# Autodesk Inventor assembly: Lime Extruder - ASM
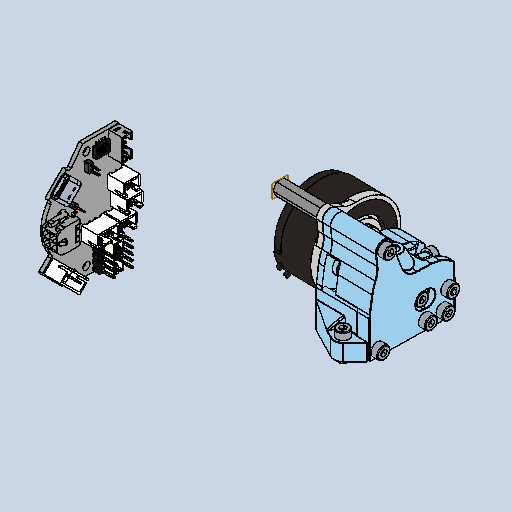
[picture p0: Inventor's stored thumbnail of the model, 512x512]
Saved by Autodesk Inventor 2026 (Build 300175050, 175E)
## iProperties
Created: 2025-07-30
Part Number: Lime Extruder - ASM
Description: STEP AP242
Document SubType Name: Assembly
Designer: tdxt
Sending System: ONSHAPE BY PTC INC, 1.201
Preprocessor: ST-DEVELOPER v20
Title: 688046dff3c7ef29f6bbb4df
## Documents named in this file (12)
- D:\Github\Lime\Lime Extruder - ASM\Lime Extruder - ASM\Lime Extruder - ASM.iam
- D:\Github\Lime\Lime Extruder - ASM\Lime Extruder - ASM\GEAR_7MM_12_TEETH_0_5_3MM_BORE.ipt
- D:\Github\Lime\Lime Extruder - ASM\Lime Extruder - ASM\Hex socket head cap screw M3x0.50 x 20.ipt
- D:\Github\Lime\Lime Extruder - ASM\Lime Extruder - ASM\Hex socket head cap screw M3x0.50 x 10.ipt
- D:\Github\Lime\Lime Extruder - ASM\Lime Extruder - ASM\Idler Arm.ipt
- D:\Github\Lime\Lime Extruder - ASM\Lime Extruder - ASM\Hex socket head cap screw M3x0.50 x 30.ipt
- D:\Github\Lime\Lime Extruder - ASM\Lime Extruder - ASM\Front Frame.ipt
- D:\Github\Lime\Lime Extruder - ASM\Lime Extruder - ASM\K1_EXTRUDER_MOTOR_-_MOONS_CSE14.ipt
- D:\Github\Lime\Lime Extruder - ASM\Lime Extruder - ASM\Back Frame.ipt
- D:\Github\Lime\Lime Extruder - ASM\hex spacer standoff nut_M3 L20\hex spacer standoff nut_M3 L20\hex spacer standoff nut_M3 L20.ipt
- D:\Github\Lime\Lime Extruder - ASM\EBB36 v4\EBB36 v4\EBB36 v4.ipt
- D:\Github\Lime\Lime Extruder - ASM\Lime Extruder - ASM\CAN Board Holder.ipt
## Components (18 placed, 17 different names)
1. Idler Arm — 旋转:6, 旋转:14
2. Front Plate — 旋转:2, 旋转:3, 旋转:7, 旋转:9, 旋转:10, 旋转:11, 旋转:12, 旋转:13
3. Back Plate — 旋转:2, 旋转:3, 旋转:4, 旋转:5, 旋转:6, 刚性:1, 旋转:8
4. EBB36 v4:1
5. CAN Board Holder:1 — 表面齐平:1
6. NAUO1 — 旋转:1
7. NAUO11 — 旋转:1, 旋转:4, 旋转:5, 插入:1, 插入:2
8. hex spacer standoff nut_M3 L20:1 — 插入:2
9. hex spacer standoff nut_M3 L20:2 — 插入:1, 表面齐平:1
10. NAUO2 — 旋转:11
11. NAUO5 — 旋转:9
12. NAUO13 — 旋转:10
13. NAUO3 — 旋转:14
14. NAUO7 — 刚性:1
15. NAUO8 — 旋转:12
16. NAUO9 — 旋转:13
17. NAUO10 — 旋转:7
18. NAUO12 — 旋转:8
## Relationships (18: RevoluteJoint 14, Insert 2, WeldJoint 1, Flush 1)
- 旋转:1 [RevoluteJoint]: NAUO1 ↔ NAUO11
- 旋转:2 [RevoluteJoint] (-0.1 mm): Front Plate ↔ Back Plate
- 旋转:3 [RevoluteJoint] (0.2 mm): Front Plate ↔ Back Plate
- 旋转:4 [RevoluteJoint]: Back Plate ↔ NAUO11
- 旋转:5 [RevoluteJoint]: Back Plate ↔ NAUO11
- 旋转:6 [RevoluteJoint] (0.2 mm): Idler Arm ↔ Back Plate
- 旋转:7 [RevoluteJoint] (3 mm): Front Plate ↔ NAUO10
- 刚性:1 [WeldJoint]: Back Plate ↔ NAUO7
- 旋转:8 [RevoluteJoint]: Back Plate ↔ NAUO12
- 旋转:9 [RevoluteJoint]: Front Plate ↔ NAUO5
- 旋转:10 [RevoluteJoint]: Front Plate ↔ NAUO13
- 旋转:11 [RevoluteJoint]: Front Plate ↔ NAUO2
- 旋转:12 [RevoluteJoint]: Front Plate ↔ NAUO8
- 旋转:13 [RevoluteJoint]: Front Plate ↔ NAUO9
- 旋转:14 [RevoluteJoint]: Idler Arm ↔ NAUO3
- 插入:1 [Insert]: NAUO11 ↔ hex spacer standoff nut_M3 L20:2
- 插入:2 [Insert]: NAUO11 ↔ hex spacer standoff nut_M3 L20:1
- 表面齐平:1 [Flush]: CAN Board Holder:1 ↔ hex spacer standoff nut_M3 L20:2
